# Autodesk Inventor assembly: SHOULDER PRINT ORIENTATION
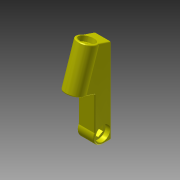
[picture p0: Inventor's stored thumbnail of the model, 180x180]
Saved by Autodesk Inventor 2013 (Build 170138000, 138)
## iProperties
Created: 2013-12-09
Part Number: SHOULDER PRINT ORIENTATION
Document SubType Name: Assembly
Designer: employee
Author: employee
## Documents named in this file (2)
- C:\Users\employee\Desktop\ConceptFORGE\ConceptFORGE\GUS Simpson\INVENTOR FILES\SHOULDER PRINT ORIENTATION.iam
- C:\Users\employee\Desktop\ConceptFORGE\ConceptFORGE\GUS Simpson\INVENTOR FILES\SHOULDER.ipt
## Components (1 placed, 1 different names)
1. SHOULDER:1 — Mate:1
## Relationships (1: Mate 1)
- Mate:1: SHOULDER:1
